# Autodesk Inventor assembly: CE-7.1.1_LS1
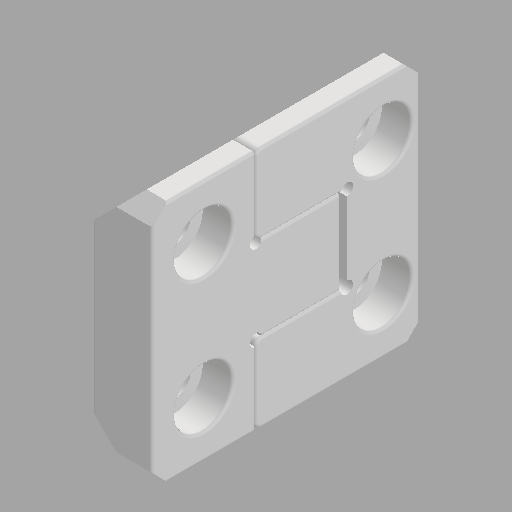
[picture p0: Inventor's stored thumbnail of the model, 512x512]
Saved by Autodesk Inventor 2024 (Build 280153000, 153)
## iProperties
Created: 2024-02-25
Part Number: CE-7.1.1_LS1
Document SubType Name: Assembly
Designer: Alex
Author: Alex
## Documents named in this file (3)
- C:\Shared\alex-bartella-schoolwork\4z03\Week 6\LS\DME_FW45 2\CE-7.1.1_LS1.iam
- C:\Shared\alex-bartella-schoolwork\4z03\Week 6\LS\DME_FW45 2\CE-7.1.1_LS1_FW45_F.ipt
- C:\Shared\alex-bartella-schoolwork\4z03\Week 6\LS\DME_FW45 2\CE-7.1.1_LS1_FW45_M.ipt
## Components (2 placed, 2 different names)
1. CE-7.1.1_LS1_FW45_F:1 — Flush:1, Flush:2, Flush:3
2. CE-7.1.1_LS1_FW45_M:1 — Flush:1, Flush:2, Flush:3, Flush:4, Flush:5, Flush:6
## Relationships (6: Flush 6)
- Flush:1: CE-7.1.1_LS1_FW45_F:1 ↔ CE-7.1.1_LS1_FW45_M:1
- Flush:2: CE-7.1.1_LS1_FW45_F:1 ↔ CE-7.1.1_LS1_FW45_M:1
- Flush:3: CE-7.1.1_LS1_FW45_F:1 ↔ CE-7.1.1_LS1_FW45_M:1
- Flush:4: CE-7.1.1_LS1_FW45_M:1
- Flush:5: CE-7.1.1_LS1_FW45_M:1
- Flush:6: CE-7.1.1_LS1_FW45_M:1
